# Autodesk Inventor assembly: Challenge Field
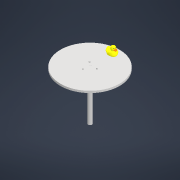
[picture p0: Inventor's stored thumbnail of the model, 180x180]
Saved by Autodesk Inventor 2022 (Build 260153000, 153)
## iProperties
Created: 2021-10-11
Part Number: Challenge Field
Document SubType Name: Assembly
Designer: zehrab
Author: zehrab
## Documents named in this file (4)
- C:\Users\zehrab\Documents\GitHub\ComputerAidedDesign\2021-22\FTC\#13822 Robovikes\Challenge Field\Challenge Field.iam
- C:\Users\zehrab\Documents\GitHub\ComputerAidedDesign\2021-22\FTC\#13822 Robovikes\Duck Carousel\Carousel Base.ipt
- C:\Users\zehrab\Documents\GitHub\ComputerAidedDesign\2021-22\FTC\#13822 Robovikes\Duck Carousel\Carousel.ipt
- C:\Users\zehrab\Documents\GitHub\ComputerAidedDesign\2021-22\FTC\#13822 Robovikes\Duck Carousel\am-4510 Rubber Duck.ipt
## Components (3 placed, 3 different names)
1. Carousel Base:1
2. Carousel:1
3. am-4510 Rubber Duck:1
## Relationships (3: Mate 2, Flush 1)
- [Mate]: Carousel Base:1 ↔ Carousel:1
- [Flush]: Carousel Base:1 ↔ Carousel:1
- [Mate]: Carousel:1 ↔ am-4510 Rubber Duck:1
